# Autodesk Inventor assembly: 0001_ASS_Ban_lap_ghep_02
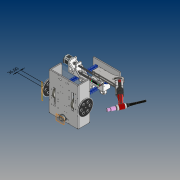
[picture p0: Inventor's stored thumbnail of the model, 180x180]
Saved by Autodesk Inventor 2021 (Build 250183000, 183)
## iProperties
Created: 2024-04-01
Part Number: 0001_ASS_Ban_lap_ghep_02
Document SubType Name: Assembly
Designer: Admin
Author: Admin
## Documents named in this file (25)
- C:\Users\Admin\Desktop\DO_AN_TOT_NGHIEP_2024\Mechanical\Design_in_3D\Version_1\0001_ASS_Ban_lap_ghep_02.iam
- C:\Users\Admin\Desktop\DO_AN_TOT_NGHIEP_2024\Mechanical\Design_in_3D\Version_1\000ASS_Bo_banh_xe_04.iam
- C:\Users\Admin\Desktop\DO_AN_TOT_NGHIEP_2024\Mechanical\Design_in_3D\Version_1\06_Tam_de_01.ipt
- C:\Users\Admin\Desktop\DO_AN_TOT_NGHIEP_2024\Mechanical\Design_in_3D\Version_1\08_Tam_canh_hong.ipt
- C:\Users\Admin\Desktop\DO_AN_TOT_NGHIEP_2024\Mechanical\Design_in_3D\Version_1\09_Tam_canh_top_bottom.ipt
- C:\Users\Admin\Desktop\DO_AN_TOT_NGHIEP_2024\Mechanical\Design_in_3D\Version_1\10_Tam_go_mat_top.ipt
- C:\Users\Admin\Desktop\Do_an\Ver_3\Thu_vien\67060-roller-ball-bearing-1.snapshot.1\67060, ROLLER BALL BEARING.iam
- C:\Users\Admin\Documents\Inventor\Content Center Files\R2021\en-US\BS EN ISO 7045 Z\EN ISO 7045 - M6 x 60 - 4.8 - Z(1).ipt
- C:\Users\Admin\Desktop\DO_AN_TOT_NGHIEP_2024\Mechanical\Design_in_3D\Library\Lo_xo_phi_7x40.ipt
- C:\Users\Admin\Desktop\DO_AN_TOT_NGHIEP_2024\Mechanical\Design_in_3D\Version_1\11_Mieng_go_dem_lo_xo.ipt
- C:\Users\Admin\Desktop\DO_AN_TOT_NGHIEP_2024\Mechanical\Design_in_3D\Version_1\12_Thong_lo_xo.ipt
- C:\Users\Admin\Desktop\DO_AN_TOT_NGHIEP_2024\Mechanical\Design_in_3D\Version_1\13_Truc_phi_10x70.ipt
- C:\Users\Admin\Desktop\DO_AN_TOT_NGHIEP_2024\Mechanical\Design_in_3D\Version_1\14_Co_dinh_cay_nen_lo_xo.ipt
- C:\Users\Admin\Desktop\DO_AN_TOT_NGHIEP_2024\Mechanical\Design_in_3D\Version_1\001_Khung_nhom.iam
- C:\Users\Admin\Desktop\DO_AN_TOT_NGHIEP_2024\Mechanical\Design_in_3D\Version_1\15_Top_truc_vit.ipt
- C:\Users\Admin\Desktop\DO_AN_TOT_NGHIEP_2024\Mechanical\Design_in_3D\Version_1\15_Khop_trung_gian.ipt
- C:\Users\Admin\Desktop\DO_AN_TOT_NGHIEP_2024\Mechanical\Design_in_3D\Version_1\002_Bo_truot.iam
- C:\Users\Admin\Desktop\DO_AN_TOT_NGHIEP_2024\Mechanical\Design_in_3D\Version_1\0012_Bo_truot.iam
- C:\Users\Admin\Desktop\DO_AN_TOT_NGHIEP_2024\Mechanical\Design_in_3D\Library\hgr-20-1.snapshot.3\Modify_KyAnh\Thanh_truot_20x200.ipt
- C:\Users\Admin\Desktop\DO_AN_TOT_NGHIEP_2024\Mechanical\Design_in_3D\Library\Vit_me_300x12.ipt
- C:\Users\Admin\Desktop\Do_an\Ver_3\Thu_vien\KFL_08_3\KFL08 - Mancal Flange oval Ø8.ipt
- C:\Users\Admin\Desktop\DO_AN_TOT_NGHIEP_2024\Mechanical\Design_in_3D\Library\stepper-motor-flexible-coupling-6-35-x-8-mm-1.snapshot.2\Stepper Motor Flexible Coupling 6,35 x 8 mm.iam
- C:\Users\Admin\Desktop\DO_AN_TOT_NGHIEP_2024\Mechanical\Design_in_3D\Library\nema-23hs5628-1.snapshot.4\NEMA_235628-6.35_s_TOP.iam
- C:\Users\Admin\Desktop\DO_AN_TOT_NGHIEP_2024\Mechanical\Design_in_3D\Version_1\16_Khau_hai.ipt
- C:\Users\Admin\Desktop\DO_AN_TOT_NGHIEP_2024\Mechanical\Design_in_3D\Version_1\21_Tam_go_trung_gian.ipt
## Components (30 placed, 24 different names)
1. 000ASS_Bo_banh_xe_04:1 [sub-assembly] — Mate:1, Mate:3, Symmetry:1
2. 000ASS_Bo_banh_xe_04:2 [sub-assembly] — Mate:2, Mate:3, Angle:1, Flush:1, Symmetry:1, Mate:4
3. 06_Tam_de_01:1 — Mate:1, Mate:2, Angle:1, Flush:1, Mate:4, Flush:2, Mate:5, Flush:3, Mate:6, Flush:4, Flush:5, Mate:7, Flush:6, Flush:7, Mate:10, Mate:25, Mate:26, Flush:11, Insert:1, Mate:29
4. 08_Tam_canh_hong:1 — Flush:2, Mate:5, Flush:3, Mate:8, Mate:12
5. 08_Tam_canh_hong:2 — Mate:6, Flush:4, Flush:5, Mate:9
6. 09_Tam_canh_top_bottom:1 — Mate:7, Flush:6, Mate:8, Flush:8, Mate:11, Mate:35, Insert:3
7. 09_Tam_canh_top_bottom:2 — Flush:7, Mate:9, Mate:10
8. 10_Tam_go_mat_top:1 — Flush:8, Mate:11, Mate:12, Mate:36, Mate:37
9. 67060, ROLLER BALL BEARING:1 [sub-assembly] — Mate:19, Mate:20, Flush:10, Flush:11
10. BS EN ISO 7045 Z - Metric M6 x 60 - 4.8 - Z:1 — Mate:19, Flush:9, Flush:10, Mate:21, Mate:25, Insert:2
11. BS EN ISO 7045 Z - Metric M6 x 60 - 4.8 - Z:2 — Mate:20, Flush:9, Mate:22, Mate:26, Mate:32
12. Lo_xo_phi_7x40:1 — Mate:22, Mate:31
13. Lo_xo_phi_7x40:2 — Mate:21, Mate:30
14. 11_Mieng_go_dem_lo_xo:1 — Insert:1, Mate:29, Mate:30, Mate:31, Mate:34
15. 12_Thong_lo_xo:1 — Mate:32, Insert:2, Mate:33
16. 13_Truc_phi_10x70:1 — Mate:33, Mate:34
17. 14_Co_dinh_cay_nen_lo_xo:1 — Mate:35, Insert:3
18. 001_Khung_nhom:1 [sub-assembly] — Mate:36, Mate:37, Mate:38, Mate:39, Flush:12, Mate:40
19. 15_Top_truc_vit:1 — Mate:38, Mate:39, Flush:12, Angle:3
20. 15_Khop_trung_gian:1 — Mate:40, Mate:41, Angle:2, Mate:47, Mate:48, Angle:3, Mate:50, Mate:51, Mate:52, Mate:54, Angle:4
21. 002_Bo_truot:1 [sub-assembly] — Mate:44, Mate:49, Mate:55, Mate:56
22. 0012_Bo_truot:1 [sub-assembly] — Mate:42, Mate:43, Mate:44, Mate:49, Mate:53, Flush:13, Insert:8
23. Thanh_truot_20x200:1 — Mate:41, Angle:2, Mate:42, Mate:43, Mate:47
24. Vit_me_300x12:1 — Insert:5, Insert:6, Mate:53
25. KFL08 - Mancal Flange oval Ø8:1 — Insert:5, Mate:51
26. KFL08 - Mancal Flange oval Ø8:2 — Insert:6, Insert:7, Mate:48, Mate:50
27. Stepper Motor Flexible Coupling 6,35 x 8 mm:1 [sub-assembly] — Insert:7
28. NEMA_235628-6.35_s_TOP:1 [sub-assembly] — Mate:52, Mate:54, Angle:4
29. 16_Khau_hai:1 — Mate:55, Flush:13, Mate:56, Mate:57
30. 21_Tam_go_trung_gian:1 — Insert:8, Mate:57
## Relationships (70: Mate 45, Flush 13, Insert 7, Angle 4, Symmetry 1)
- Mate:1: 000ASS_Bo_banh_xe_04:1 ↔ 06_Tam_de_01:1
- Mate:2: 000ASS_Bo_banh_xe_04:2 ↔ 06_Tam_de_01:1
- Mate:3: 000ASS_Bo_banh_xe_04:1 ↔ 000ASS_Bo_banh_xe_04:2
- Angle:1 (0 deg): 000ASS_Bo_banh_xe_04:2 ↔ 06_Tam_de_01:1
- Flush:1 (15 mm): 000ASS_Bo_banh_xe_04:2 ↔ 06_Tam_de_01:1
- Symmetry:1: 000ASS_Bo_banh_xe_04:1 ↔ 000ASS_Bo_banh_xe_04:2
- Mate:4: 000ASS_Bo_banh_xe_04:2 ↔ 06_Tam_de_01:1
- Flush:2: 06_Tam_de_01:1 ↔ 08_Tam_canh_hong:1
- Mate:5: 06_Tam_de_01:1 ↔ 08_Tam_canh_hong:1
- Flush:3: 06_Tam_de_01:1 ↔ 08_Tam_canh_hong:1
- Mate:6: 06_Tam_de_01:1 ↔ 08_Tam_canh_hong:2
- Flush:4: 06_Tam_de_01:1 ↔ 08_Tam_canh_hong:2
- Flush:5: 06_Tam_de_01:1 ↔ 08_Tam_canh_hong:2
- Mate:7: 06_Tam_de_01:1 ↔ 09_Tam_canh_top_bottom:1
- Flush:6: 06_Tam_de_01:1 ↔ 09_Tam_canh_top_bottom:1
- Mate:8: 08_Tam_canh_hong:1 ↔ 09_Tam_canh_top_bottom:1
- Flush:7: 06_Tam_de_01:1 ↔ 09_Tam_canh_top_bottom:2
- Mate:9: 08_Tam_canh_hong:2 ↔ 09_Tam_canh_top_bottom:2
- Mate:10: 06_Tam_de_01:1 ↔ 09_Tam_canh_top_bottom:2
- Flush:8: 09_Tam_canh_top_bottom:1 ↔ 10_Tam_go_mat_top:1
- Mate:11: 09_Tam_canh_top_bottom:1 ↔ 10_Tam_go_mat_top:1
- Mate:12: 08_Tam_canh_hong:1 ↔ 10_Tam_go_mat_top:1
- Mate:19: 67060, ROLLER BALL BEARING:1 ↔ BS EN ISO 7045 Z - Metric M6 x 60 - 4.8 - Z:1
- Mate:20: 67060, ROLLER BALL BEARING:1 ↔ BS EN ISO 7045 Z - Metric M6 x 60 - 4.8 - Z:2
- Flush:9: BS EN ISO 7045 Z - Metric M6 x 60 - 4.8 - Z:1 ↔ BS EN ISO 7045 Z - Metric M6 x 60 - 4.8 - Z:2
- Flush:10: 67060, ROLLER BALL BEARING:1 ↔ BS EN ISO 7045 Z - Metric M6 x 60 - 4.8 - Z:1
- Mate:21: BS EN ISO 7045 Z - Metric M6 x 60 - 4.8 - Z:1 ↔ Lo_xo_phi_7x40:2
- Mate:22: BS EN ISO 7045 Z - Metric M6 x 60 - 4.8 - Z:2 ↔ Lo_xo_phi_7x40:1
- Mate:25: 06_Tam_de_01:1 ↔ BS EN ISO 7045 Z - Metric M6 x 60 - 4.8 - Z:1
- Mate:26: 06_Tam_de_01:1 ↔ BS EN ISO 7045 Z - Metric M6 x 60 - 4.8 - Z:2
- Flush:11 (-33 mm): 06_Tam_de_01:1 ↔ 67060, ROLLER BALL BEARING:1
- Insert:1: 06_Tam_de_01:1 ↔ 11_Mieng_go_dem_lo_xo:1
- Mate:29: 06_Tam_de_01:1 ↔ 11_Mieng_go_dem_lo_xo:1
- Mate:30: Lo_xo_phi_7x40:2 ↔ 11_Mieng_go_dem_lo_xo:1
- Mate:31: Lo_xo_phi_7x40:1 ↔ 11_Mieng_go_dem_lo_xo:1
- Mate:32: BS EN ISO 7045 Z - Metric M6 x 60 - 4.8 - Z:2 ↔ 12_Thong_lo_xo:1
- Insert:2: BS EN ISO 7045 Z - Metric M6 x 60 - 4.8 - Z:1 ↔ 12_Thong_lo_xo:1
- Mate:33: 12_Thong_lo_xo:1 ↔ 13_Truc_phi_10x70:1
- Mate:34: 11_Mieng_go_dem_lo_xo:1 ↔ 13_Truc_phi_10x70:1
- Mate:35: 09_Tam_canh_top_bottom:1 ↔ 14_Co_dinh_cay_nen_lo_xo:1
- Insert:3: 09_Tam_canh_top_bottom:1 ↔ 14_Co_dinh_cay_nen_lo_xo:1
- Mate:36: 10_Tam_go_mat_top:1 ↔ 001_Khung_nhom:1
- Mate:37: 10_Tam_go_mat_top:1 ↔ 001_Khung_nhom:1
- Mate:38: 001_Khung_nhom:1 ↔ 15_Top_truc_vit:1
- Mate:39: 001_Khung_nhom:1 ↔ 15_Top_truc_vit:1
- Flush:12: 001_Khung_nhom:1 ↔ 15_Top_truc_vit:1
- Mate:40: 001_Khung_nhom:1 ↔ 15_Khop_trung_gian:1
- Mate:41: 15_Khop_trung_gian:1 ↔ Thanh_truot_20x200:1
- Angle:2 (0 deg): 15_Khop_trung_gian:1 ↔ Thanh_truot_20x200:1
- Mate:42: 0012_Bo_truot:1 ↔ Thanh_truot_20x200:1
- Mate:43: 0012_Bo_truot:1 ↔ Thanh_truot_20x200:1
- Mate:44: 002_Bo_truot:1 ↔ 0012_Bo_truot:1
- Insert:5: Vit_me_300x12:1 ↔ KFL08 - Mancal Flange oval Ø8:1
- Insert:6: Vit_me_300x12:1 ↔ KFL08 - Mancal Flange oval Ø8:2
- Insert:7 (2 mm): KFL08 - Mancal Flange oval Ø8:2 ↔ Stepper Motor Flexible Coupling 6,35 x 8 mm:1
- Mate:47: 15_Khop_trung_gian:1 ↔ Thanh_truot_20x200:1
- Mate:48: 15_Khop_trung_gian:1 ↔ KFL08 - Mancal Flange oval Ø8:2
- Angle:3 (180 deg): 15_Top_truc_vit:1 ↔ 15_Khop_trung_gian:1
- Mate:49: 002_Bo_truot:1 ↔ 0012_Bo_truot:1
- Mate:50: 15_Khop_trung_gian:1 ↔ KFL08 - Mancal Flange oval Ø8:2
- Mate:51: 15_Khop_trung_gian:1 ↔ KFL08 - Mancal Flange oval Ø8:1
- Mate:52: 15_Khop_trung_gian:1 ↔ NEMA_235628-6.35_s_TOP:1
- Mate:53: 0012_Bo_truot:1 ↔ Vit_me_300x12:1
- Mate:54: 15_Khop_trung_gian:1 ↔ NEMA_235628-6.35_s_TOP:1
- Angle:4 (0 deg): 15_Khop_trung_gian:1 ↔ NEMA_235628-6.35_s_TOP:1
- Mate:55: 002_Bo_truot:1 ↔ 16_Khau_hai:1
- Flush:13: 0012_Bo_truot:1 ↔ 16_Khau_hai:1
- Mate:56: 002_Bo_truot:1 ↔ 16_Khau_hai:1
- Insert:8: 0012_Bo_truot:1 ↔ 21_Tam_go_trung_gian:1
- Mate:57: 16_Khau_hai:1 ↔ 21_Tam_go_trung_gian:1
